# Autodesk Inventor assembly: Version 1
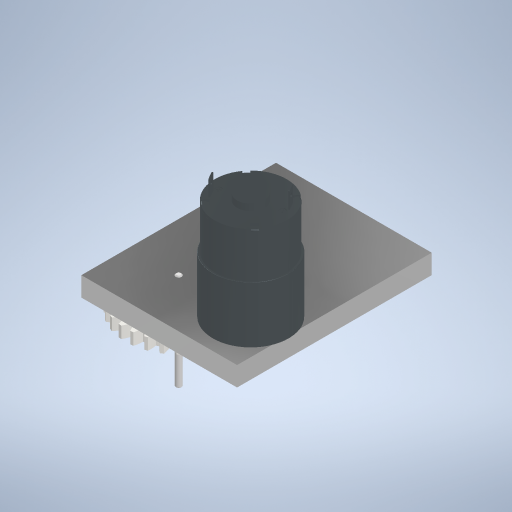
[picture p0: Inventor's stored thumbnail of the model, 512x512]
Saved by Autodesk Inventor 2024.2 (Build 282272000, 272)
## iProperties
Created: 2024-03-11
Part Number: Version 1
Document SubType Name: Assembly
Designer: evmgm
Author: evmgm
## Documents named in this file (5)
- C:\Users\evmgm\OneDrive - Syddansk Universitet\SDU OneDrive\2. Semester\Semerster projekt 2\Version 1.iam
- C:\Users\evmgm\OneDrive - Syddansk Universitet\SDU OneDrive\2. Semester\Semerster projekt 2\Support test1.ipt
- C:\Users\evmgm\OneDrive - Syddansk Universitet\SDU OneDrive\2. Semester\Semerster projekt 2\moteur_NIDEC_HG37-120-AB-00__HG37-150-AB-00__HG37-200-AB-00__HG37-300-AB-00\moteur_NIDEC_HG37-120-AB-00__HG37-150-AB-0.ipt
- C:\Users\evmgm\OneDrive - Syddansk Universitet\SDU OneDrive\2. Semester\Semerster projekt 2\3mm Shaft50.ipt
- C:\Users\evmgm\OneDrive - Syddansk Universitet\SDU OneDrive\2. Semester\Semerster projekt 2\Version 1\Design Accelerator\Spur Gears2.iam
## Components (5 placed, 4 different names)
1. Support test1:1 — Rigid:2, Rigid:3, Mate:2, Mate:4, Rigid:4
2. moteur_NIDEC_HG37-120-AB-00__HG37-150-AB-0:1 — Rigid:4
3. 3mm Shaft50:1 — Rigid:3, Mate:1
4. 3mm Shaft50:2 — Rigid:2, Mate:3
5. Spur Gears:1 [sub-assembly] — Mate:1, Mate:2, Mate:3, Mate:4
## Relationships (7: Mate 4, WeldJoint 3)
- Rigid:2 [WeldJoint]: Support test1:1 ↔ 3mm Shaft50:2
- Rigid:3 [WeldJoint]: Support test1:1 ↔ 3mm Shaft50:1
- Mate:1: 3mm Shaft50:1 ↔ Spur Gears:1
- Mate:2: Support test1:1 ↔ Spur Gears:1
- Mate:3: 3mm Shaft50:2 ↔ Spur Gears:1
- Mate:4: Support test1:1 ↔ Spur Gears:1
- Rigid:4 [WeldJoint]: Support test1:1 ↔ moteur_NIDEC_HG37-120-AB-00__HG37-150-AB-0:1
